# Autodesk Inventor assembly: SnowBlowerMotorAndMount
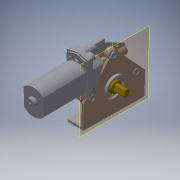
[picture p0: Inventor's stored thumbnail of the model, 180x180]
Saved by Autodesk Inventor 2016 SP1 (Build 200210100, 210)
## iProperties
Created: 2016-02-07
Part Number: SnowBlowerMotorAndMount
Document SubType Name: Assembly
Designer: steele
Author: steele
## Documents named in this file (3)
- C:\snobotics\CAD-Development\robSteele\SnoBotics2016\AM Parts\SnowBlowerMotorAndMount.iam
- C:\snobotics\CAD-Development\robSteele\SnoBotics2016\AM Parts\rsSnowBlowerMount.ipt
- C:\snobotics\CAD-Development\robSteele\SnoBotics2016\AM Parts\SnowBlowerMotor.iam
## Components (2 placed, 2 different names)
1. rsSnowBlowerMount:1 — Insert:1, Flush:1
2. SnowBlowerMotor:1 [sub-assembly] — Insert:1
## Relationships (2: Insert 1, Flush 1)
- Insert:1: rsSnowBlowerMount:1 ↔ SnowBlowerMotor:1
- Flush:1: rsSnowBlowerMount:1
